# Autodesk Inventor assembly: CCM_Base_Mount
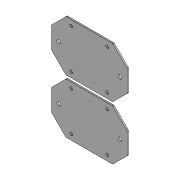
[picture p0: Inventor's stored thumbnail of the model, 180x180]
Saved by Autodesk Inventor 2020 (Build 240168000, 168)
## iProperties
Created: 2021-07-28
Part Number: CCM_Base_Mount
Document SubType Name: Assembly
Designer: magnarecta
Author: magnarecta
## Documents named in this file (2)
- C:\Users\lvglv\Documents\GitHub\Eto_Project\Hardware\Parts\Meviy\Meviy_Asem\CCM_Base_Mount.iam
- C:\Users\lvglv\Documents\GitHub\Eto_Project\Hardware\Parts\Meviy\CCM_Mount_C.ipt
## Components (2 placed, 1 different names)
1. CCM_Mount_C:1 — フラッシュ:1, フラッシュ:2, メイト:1
2. CCM_Mount_C:2 — フラッシュ:1, フラッシュ:2, メイト:1
## Relationships (3: Flush 2, Mate 1)
- フラッシュ:1 [Flush]: CCM_Mount_C:1 ↔ CCM_Mount_C:2
- フラッシュ:2 [Flush]: CCM_Mount_C:1 ↔ CCM_Mount_C:2
- メイト:1 [Mate] (5 mm): CCM_Mount_C:1 ↔ CCM_Mount_C:2
